# Autodesk Inventor assembly: drivebay_MIR
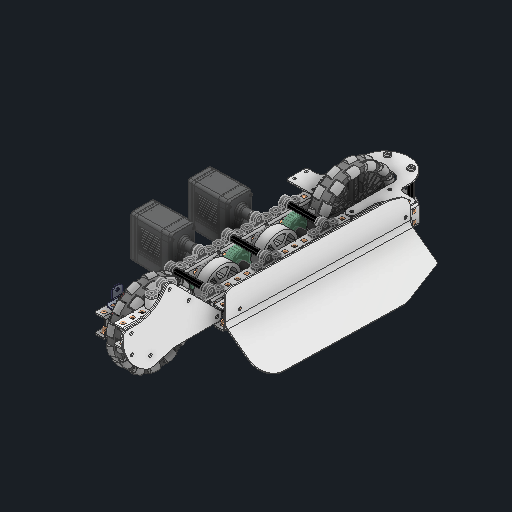
[picture p0: Inventor's stored thumbnail of the model, 512x512]
Saved by Autodesk Inventor 2024 (Build 280153000, 153)
## iProperties
Created: 2023-08-15
Part Number: drivebay_MIR
Document SubType Name: Assembly
Designer: avere
Author: avere
## Documents named in this file (25)
- D:\vex_robotics\hardware\cad\spades_v0.1\chassis\mirrored_parts\drivebay_MIR.iam
- D:\vex_robotics\hardware\cad\spades_v0.1\chassis\mirrored_parts\outer_MIR.iam
- D:\vex_robotics\hardware\cad\spades_v0.1\chassis\mirrored_parts\inner_MIR.iam
- D:\vex_robotics\hardware\cad\spades_v0.1\chassis\mirrored_parts\wheel_MIR.iam
- D:\vex_robotics\hardware\cad\spades_v0.1\chassis\mirrored_parts\gear_MIR.iam
- D:\vex_robotics\hardware\cad\spades_v0.1\chassis\mirrored_parts\gusset_MIR.ipt
- D:\vex_robotics\hardware\cad\VEX-CAD-Inventor-1.41\Motion\Spacers\Spacer Nylon .500 OD\NSpacer White .500 OD x .500.ipt
- D:\vex_robotics\hardware\cad\VEX-CAD-Inventor-1.41\Structure\Standoff\Standoff 1.50.ipt
- D:\vex_robotics\hardware\cad\VEX-CAD-Inventor-1.41\Motion\Spacers\Spacer Nylon .375 OD\NSpacer .375 OD x .125.ipt
- D:\vex_robotics\hardware\cad\spades_v0.1\chassis\custom_parts\sled.ipt
- D:\vex_robotics\hardware\cad\VEX-CAD-Inventor-1.41\Structure\C Channel\Aluminum 1x2x1\Alu C 1x2x1x7.ipt
- D:\vex_robotics\hardware\cad\spades_v0.1\chassis\mirrored_parts\flapper_MIR.iam
- D:\vex_robotics\hardware\cad\VEX-CAD-Inventor-1.41\Motion\Spacers\Spacer Nylon .375 OD\NSpacer .375 OD x .375.ipt
- D:\vex_robotics\hardware\cad\VEX-CAD-Inventor-1.41\Motion\Spacers\Washer Steel\SWasher .375 OD x .062500.ipt
- D:\vex_robotics\hardware\cad\VEX-CAD-Inventor-1.41\Motion\Spacers\Washer Steel\SWasher .375 OD x .015625.ipt
- D:\vex_robotics\hardware\cad\VEX-CAD-Inventor-1.41\Motion\Spacers\Washer Teflon\TWasher .375 OD x .04000.ipt
- D:\vex_robotics\hardware\cad\spades_v0.1\chassis\flex_wheel.iam
- D:\vex_robotics\hardware\cad\VEX-CAD-Inventor-1.41\Motion\Shaft LS\LS Pillow Bearing Block.ipt
- D:\vex_robotics\hardware\cad\hardware\Nylon Screw Pan-Head .375.ipt
- D:\vex_robotics\hardware\cad\VEX-CAD-Inventor-1.41\Motion\Spacers\Spacer Nylon .500 OD.ipt
- D:\vex_robotics\hardware\cad\VEX-CAD-Inventor-1.41\Structure\Standoff.ipt
- D:\vex_robotics\hardware\cad\VEX-CAD-Inventor-1.41\Motion\Spacers\Spacer Nylon .375 OD.ipt
- D:\vex_robotics\hardware\cad\VEX-CAD-Inventor-1.41\Motion\Spacers\Washer Steel.ipt
- D:\vex_robotics\hardware\cad\VEX-CAD-Inventor-1.41\Motion\Spacers\Washer Teflon.ipt
- D:\vex_robotics\hardware\cad\VEX-CAD-Inventor-1.41\Motion\Shaft LS\Shaft Collar ipts\Shaft Collar Set Screw.ipt
## Components (44 placed, 19 different names)
1. outer_MIR:1 [sub-assembly] — Insert:3, Insert:4, Insert:27, Mate:5, Mate:6, Insert:30, Insert:32, Insert:34, Insert:35, Insert:36, Insert:42, Insert:43
2. inner_MIR:1 [sub-assembly] — Mate:3, Insert:10, Mate:4, Insert:11, Insert:12, Insert:20, Mate:9, Mate:10, Insert:53
3. wheel_MIR:1 [sub-assembly] — Insert:3
4. wheel_MIR:2 [sub-assembly] — Insert:4
5. gear_MIR:1 [sub-assembly] — Insert:30
6. gear_MIR:2 [sub-assembly] — Insert:34
7. gear_MIR:5 [sub-assembly] — Insert:32
8. gusset_MIR:1 — Mate:3, Insert:10, Insert:17, Insert:16, Insert:37, Insert:49, Insert:50
9. gusset_MIR:2 — Mate:4, Insert:11, Insert:13, Insert:14, Insert:15, Insert:51, Insert:52
10. NSpacer White .500 OD x .500:1 — Insert:12
11. NSpacer White .500 OD x .500:2 — Insert:13
12. NSpacer White .500 OD x .500:3 — Insert:14
13. NSpacer White .500 OD x .500:4 — Insert:15
14. Standoff 1.50:1 — Insert:17
15. Standoff 1.50:2 — Insert:16
16. Standoff 1.50:3 — Insert:18, Insert:19
17. NSpacer .375 OD x .125:1 — Insert:18
18. NSpacer .375 OD x .125:2 — Insert:20, Insert:19
19. Standoff 1.50:4 — Insert:21, Insert:22
20. NSpacer .375 OD x .125:3 — Insert:21, Mate:9
21. NSpacer .375 OD x .125:4 — Insert:22, Insert:36
22. Standoff 1.50:5 — Insert:24, Insert:25
23. NSpacer .375 OD x .125:5 — Insert:24, Mate:10
24. NSpacer .375 OD x .125:6 — Insert:25, Insert:35
25. sled:1 — Insert:28, Mate:6, Insert:29, Mate:7, Insert:48
26. Alu C 1x2x1x7:1 — Insert:27, Mate:5, Insert:28, Insert:44, Insert:46
27. sled:2 — Insert:29, Mate:7
28. flapper_MIR:1 [sub-assembly] — Insert:37, Insert:41
29. NSpacer .375 OD x .375:7 — Insert:41
30. SWasher .375 OD x .062500:1
31. SWasher .375 OD x .015625:2
32. TWasher .375 OD x .04000:1
33. flex_wheel:1 [sub-assembly] — Insert:42
34. flex_wheel:2 [sub-assembly] — Insert:43
35. LS Pillow Bearing Block:1 — Insert:45, Mate:8
36. NSpacer White .500 OD x .500:5 — Insert:44, Insert:45
37. NSpacer White .500 OD x .500:6 — Insert:46, Mate:8
38. NSpacer .375 OD x .125:8 — Insert:47
39. SWasher .375 OD x .062500:3 — Insert:47, Insert:48
40. Nylon Screw Pan-Head .375:1 — Insert:49
41. Nylon Screw Pan-Head .375:2 — Insert:50
42. Nylon Screw Pan-Head .375:3 — Insert:51
43. Nylon Screw Pan-Head .375:4 — Insert:52
44. Shaft Collar Set Screw:1 — Insert:53
## Relationships (50: Insert 42, Mate 8)
- Insert:3 (13.716 mm): outer_MIR:1 ↔ wheel_MIR:1
- Insert:4 (13.716 mm): outer_MIR:1 ↔ wheel_MIR:2
- Mate:3: inner_MIR:1 ↔ gusset_MIR:1
- Insert:10: inner_MIR:1 ↔ gusset_MIR:1
- Mate:4: inner_MIR:1 ↔ gusset_MIR:2
- Insert:11 (12.7 mm): inner_MIR:1 ↔ gusset_MIR:2
- Insert:12: inner_MIR:1 ↔ NSpacer White .500 OD x .500:1
- Insert:13: gusset_MIR:2 ↔ NSpacer White .500 OD x .500:2
- Insert:14: gusset_MIR:2 ↔ NSpacer White .500 OD x .500:3
- Insert:15: gusset_MIR:2 ↔ NSpacer White .500 OD x .500:4
- Insert:17: gusset_MIR:1 ↔ Standoff 1.50:1
- Insert:16: gusset_MIR:1 ↔ Standoff 1.50:2
- Insert:18: Standoff 1.50:3 ↔ NSpacer .375 OD x .125:1
- Insert:20: inner_MIR:1 ↔ NSpacer .375 OD x .125:2
- Insert:19: Standoff 1.50:3 ↔ NSpacer .375 OD x .125:2
- Insert:21: Standoff 1.50:4 ↔ NSpacer .375 OD x .125:3
- Insert:22: Standoff 1.50:4 ↔ NSpacer .375 OD x .125:4
- Insert:24: Standoff 1.50:5 ↔ NSpacer .375 OD x .125:5
- Insert:25: Standoff 1.50:5 ↔ NSpacer .375 OD x .125:6
- Insert:27: outer_MIR:1 ↔ Alu C 1x2x1x7:1
- Mate:5: outer_MIR:1 ↔ Alu C 1x2x1x7:1
- Insert:28: sled:1 ↔ Alu C 1x2x1x7:1
- Mate:6: outer_MIR:1 ↔ sled:1
- Insert:29: sled:1 ↔ sled:2
- Mate:7: sled:1 ↔ sled:2
- Insert:30 (1.27 mm): outer_MIR:1 ↔ gear_MIR:1
- Insert:32 (1.27 mm): outer_MIR:1 ↔ gear_MIR:5
- Insert:34 (1.27 mm): outer_MIR:1 ↔ gear_MIR:2
- Insert:35: outer_MIR:1 ↔ NSpacer .375 OD x .125:6
- Insert:36: outer_MIR:1 ↔ NSpacer .375 OD x .125:4
- Insert:37: gusset_MIR:1 ↔ flapper_MIR:1
- [Insert]: SWasher .375 OD x .062500:1 ↔ TWasher .375 OD x .04000:1
- [Insert]: SWasher .375 OD x .015625:2 ↔ TWasher .375 OD x .04000:1
- [Insert]: NSpacer .375 OD x .375:7 ↔ SWasher .375 OD x .062500:1
- Insert:41: flapper_MIR:1 ↔ NSpacer .375 OD x .375:7
- Insert:42 (1.27 mm): outer_MIR:1 ↔ flex_wheel:1
- Insert:43 (1.27 mm): outer_MIR:1 ↔ flex_wheel:2
- Insert:44: Alu C 1x2x1x7:1 ↔ NSpacer White .500 OD x .500:5
- Insert:45: LS Pillow Bearing Block:1 ↔ NSpacer White .500 OD x .500:5
- Insert:46: Alu C 1x2x1x7:1 ↔ NSpacer White .500 OD x .500:6
- Mate:8: LS Pillow Bearing Block:1 ↔ NSpacer White .500 OD x .500:6
- Insert:47: NSpacer .375 OD x .125:8 ↔ SWasher .375 OD x .062500:3
- Insert:48: sled:1 ↔ SWasher .375 OD x .062500:3
- Mate:9: inner_MIR:1 ↔ NSpacer .375 OD x .125:3
- Mate:10: inner_MIR:1 ↔ NSpacer .375 OD x .125:5
- Insert:49: gusset_MIR:1 ↔ Nylon Screw Pan-Head .375:1
- Insert:50: gusset_MIR:1 ↔ Nylon Screw Pan-Head .375:2
- Insert:51: gusset_MIR:2 ↔ Nylon Screw Pan-Head .375:3
- Insert:52: gusset_MIR:2 ↔ Nylon Screw Pan-Head .375:4
- Insert:53: inner_MIR:1 ↔ Shaft Collar Set Screw:1
